# Autodesk Inventor assembly: Robot_Rev3
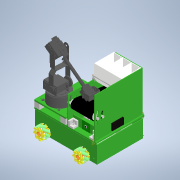
[picture p0: Inventor's stored thumbnail of the model, 180x180]
Saved by Autodesk Inventor 2020 (Build 240168000, 168)
## iProperties
Created: 2021-12-14
Part Number: Robot_Rev3
Document SubType Name: Assembly
Designer: danie
Author: danie
## Documents named in this file (15)
- C:\Users\danie\Documents\Capstone\Solidworks\Robot_Rev3.iam
- C:\Users\danie\Documents\Capstone\Solidworks\Lower Chassis_2.ipt
- C:\Users\danie\Documents\Capstone\Solidworks\UpperChassis_Base_2.ipt
- C:\Users\danie\Documents\Capstone\Solidworks\AL5D_2017_12_17.iam
- C:\Users\danie\Documents\Capstone\Solidworks\MECHANUM WHEEL.iam
- C:\Users\danie\Documents\Capstone\Solidworks\TurntableandBase.iam
- C:\Users\danie\Documents\Capstone\Solidworks\BeadCompartments_5.ipt
- C:\Users\danie\Documents\Capstone\Solidworks\False_Bottom_Geared_2.iam
- C:\Users\danie\Documents\Capstone\Solidworks\ShootingMech_Detailed2.iam
- C:\Users\danie\Documents\Capstone\Solidworks\ShootingMech_Motor.ipt
- C:\Users\danie\Documents\Capstone\Solidworks\Nav_Camera.ipt
- C:\Users\danie\Documents\Capstone\Solidworks\Periph_Screen.ipt
- C:\Users\danie\Documents\Capstone\Solidworks\Drivetrain_Motor.ipt
- C:\Users\danie\Documents\Capstone\Solidworks\MountingBracket_2.ipt
- C:\Users\danie\Documents\Capstone\Solidworks\MountingBracket_3.ipt
## Components (27 placed, 14 different names)
1. Lower Chassis_2:1 — Rigid:12, Rigid:13, Rigid:14, Rigid:15
2. UpperChassis_Base_2:1 — Rigid:5
3. AL5D_2017_12_17:1 [sub-assembly]
4. MECHANUM WHEEL:1 [sub-assembly] — Rigid:8
5. MECHANUM WHEEL:2 [sub-assembly] — Rigid:9
6. MECHANUM WHEEL:3 [sub-assembly] — Rigid:11
7. MECHANUM WHEEL:4 [sub-assembly] — Rigid:10
8. TurntableandBase:1 [sub-assembly]
9. BeadCompartments_5:1 — Rigid:2, Rigid:4
10. False_Bottom_Geared_2:1 [sub-assembly] — Rigid:2
11. ShootingMech_Detailed2:1 [sub-assembly] — Rigid:4, Rigid:5, Rigid:16
12. ShootingMech_Motor:1
13. Nav_Camera:1 — Rigid:16
14. Nav_Camera:2
15. Periph_Screen:1
16. Drivetrain_Motor:1 — Rigid:10
17. Drivetrain_Motor:2 — Rigid:11
18. Drivetrain_Motor:3 — Rigid:9
19. Drivetrain_Motor:4 — Rigid:8
20. MountingBracket_2:1 — Rigid:15
21. MountingBracket_2:2 — Rigid:14
22. MountingBracket_2:3 — Rigid:13
23. MountingBracket_2:4 — Rigid:12
24. MountingBracket_2:5
25. MountingBracket_3:1
26. MountingBracket_3:2
27. MountingBracket_3:3
## Relationships (12: WeldJoint 12)
- Rigid:2 [WeldJoint]: BeadCompartments_5:1 ↔ False_Bottom_Geared_2:1
- Rigid:4 [WeldJoint]: BeadCompartments_5:1 ↔ ShootingMech_Detailed2:1
- Rigid:5 [WeldJoint] (-6.35 mm): UpperChassis_Base_2:1 ↔ ShootingMech_Detailed2:1
- Rigid:8 [WeldJoint] (1.27 mm): MECHANUM WHEEL:1 ↔ Drivetrain_Motor:4
- Rigid:9 [WeldJoint] (-1.27 mm): MECHANUM WHEEL:2 ↔ Drivetrain_Motor:3
- Rigid:10 [WeldJoint] (-1.27 mm): MECHANUM WHEEL:4 ↔ Drivetrain_Motor:1
- Rigid:11 [WeldJoint] (-1.27 mm): MECHANUM WHEEL:3 ↔ Drivetrain_Motor:2
- Rigid:12 [WeldJoint]: Lower Chassis_2:1 ↔ MountingBracket_2:4
- Rigid:13 [WeldJoint]: Lower Chassis_2:1 ↔ MountingBracket_2:3
- Rigid:14 [WeldJoint]: Lower Chassis_2:1 ↔ MountingBracket_2:2
- Rigid:15 [WeldJoint]: Lower Chassis_2:1 ↔ MountingBracket_2:1
- Rigid:16 [WeldJoint]: ShootingMech_Detailed2:1 ↔ Nav_Camera:1
